# Autodesk Inventor assembly: LCD Mount 2 HSI
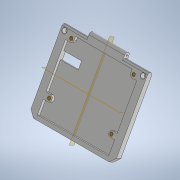
[picture p0: Inventor's stored thumbnail of the model, 180x180]
Saved by Autodesk Inventor 2022 (Build 260153000, 153)
## iProperties
Created: 2022-04-02
Part Number: LCD Mount 2 HSI
Document SubType Name: Assembly
Designer: Nick
Author: Nick
## Documents named in this file (3)
- Y:\Projects\Bibble0\3D printed\LCD Mount 2 HSI.iam
- Y:\Projects\Bibble0\3D printed\LCD Mount 2.ipt
- Y:\Projects\Bibble0\Hardware\M3 Heat Set Inserts.ipt
## Components (5 placed, 2 different names)
1. LCD Mount 2:1 — Insert:1, Insert:2, Insert:3, Insert:4
2. M3 Heat Set Inserts:1 — Insert:4
3. M3 Heat Set Inserts:2 — Insert:3
4. M3 Heat Set Inserts:3 — Insert:2
5. M3 Heat Set Inserts:4 — Insert:1
## Relationships (4: Insert 4)
- Insert:1: LCD Mount 2:1 ↔ M3 Heat Set Inserts:4
- Insert:2: LCD Mount 2:1 ↔ M3 Heat Set Inserts:3
- Insert:3: LCD Mount 2:1 ↔ M3 Heat Set Inserts:2
- Insert:4: LCD Mount 2:1 ↔ M3 Heat Set Inserts:1
